# Autodesk Inventor assembly: gearbox_MIR
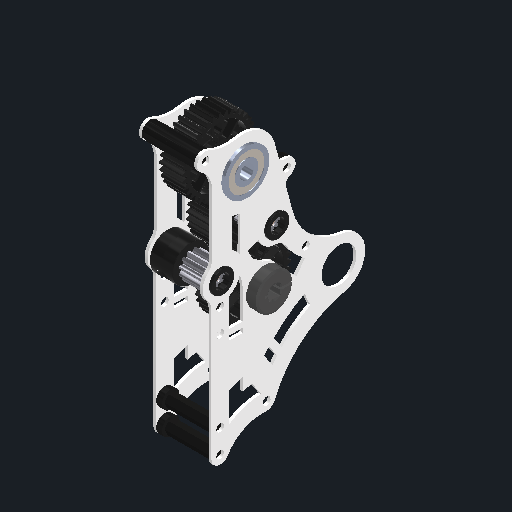
[picture p0: Inventor's stored thumbnail of the model, 512x512]
Saved by Autodesk Inventor 2024 (Build 280153000, 153)
## iProperties
Created: 2023-11-21
Part Number: gearbox_MIR
Document SubType Name: Assembly
Designer: avere
Author: avere
## Documents named in this file (14)
- C:\Users\avere\Documents\rbp_cad\zoomba_v0.1\arm\mirrored_parts\gearbox_MIR.iam
- C:\Users\avere\Documents\rbp_cad\zoomba_v0.1\arm\mirrored_parts\reservoir_mount_MIR.ipt
- C:\Users\avere\Documents\rbp_cad\zoomba_v0.1\arm\mirrored_parts\HS Bushing 0.1250_MIR.ipt
- C:\Users\avere\Documents\rbp_cad\zoomba_v0.1\arm\mirrored_parts\HS 12T Gear, No Insert_MIR.iam
- C:\Users\avere\Documents\rbp_cad\zoomba_v0.1\arm\mirrored_parts\HS 36T Gear, No Insert_MIR.iam
- C:\Users\avere\Documents\rbp_cad\zoomba_v0.1\arm\mirrored_parts\Ball Bearing_MIR.ipt
- C:\Users\avere\Documents\rbp_cad\VEX-CAD-Inventor-1.41\Structure\Standoff\Standoff 1.00.ipt
- C:\Users\avere\Documents\rbp_cad\VEX-CAD-Inventor-1.41\Structure\Standoff.ipt
- C:\Users\avere\Documents\rbp_cad\VEX-CAD-Inventor-1.41\Motion\Spacers\Spacer Nylon .375 OD\NSpacer .375 OD x .125.ipt
- C:\Users\avere\Documents\rbp_cad\VEX-CAD-Inventor-1.41\Motion\Spacers\Spacer Nylon .375 OD.ipt
- C:\Users\avere\Documents\rbp_cad\zoomba_v0.1\arm\mirrored_parts\Low Profile HS Shaft Collar_MIR.ipt
- C:\Users\avere\Documents\rbp_cad\zoomba_v0.1\arm\mirrored_parts\HS Shaft Collar_MIR.ipt
- C:\Users\avere\Documents\rbp_cad\zoomba_v0.1\arm\mirrored_parts\reservoir_mount_inner_MIR.ipt
- C:\Users\avere\Documents\rbp_cad\VEX-CAD-Inventor-1.41\Motion\Spacers\Spacer Nylon .375 OD\NSpacer .375 OD x .500.ipt
## Components (26 placed, 11 different names)
1. reservoir_mount_MIR:1 — Insert:3, Insert:1, Insert:2, Insert:17, Insert:11, Insert:13, Insert:15, Mate:1, Insert:26
2. HS Bushing 0.1250_MIR:1 — Insert:3, Insert:4
3. HS Bushing 0.1250_MIR:2 — Insert:1, Insert:5, Insert:18
4. HS Bushing 0.1250_MIR:3 — Insert:2, Insert:7
5. HS 12T Gear, No Insert_MIR:1 [sub-assembly] — Insert:4
6. HS 12T Gear, No Insert_MIR:2 [sub-assembly] — Insert:6
7. HS 36T Gear, No Insert_MIR:1 [sub-assembly] — Insert:6, Insert:5
8. HS 36T Gear, No Insert_MIR:2 [sub-assembly] — Insert:7, Insert:9
9. HS 12T Gear, No Insert_MIR:3 [sub-assembly] — Insert:9
10. Ball Bearing_MIR:1 — Insert:17
11. Standoff 1.00:1 — Insert:10
12. NSpacer .375 OD x .125:1 — Insert:11, Insert:10
13. NSpacer .375 OD x .125:2 — Insert:13, Insert:21
14. Standoff 1.00:3 — Insert:14
15. NSpacer .375 OD x .125:3 — Insert:14, Insert:15
16. HS 36T Gear, No Insert_MIR:3 [sub-assembly] — Insert:21
17. Low Profile HS Shaft Collar_MIR:1 — Insert:18
18. HS Shaft Collar_MIR:1
19. reservoir_mount_inner_MIR:1 — Mate:1, Insert:20, Insert:24, Insert:25, Insert:26
20. Ball Bearing_MIR:2 — Insert:21, Insert:20
21. NSpacer .375 OD x .500:4
22. NSpacer .375 OD x .500:5 — Insert:21
23. Standoff 1.00:4
24. NSpacer .375 OD x .125:6 — Insert:25
25. Standoff 1.00:5
26. NSpacer .375 OD x .125:7 — Insert:24
## Relationships (25: Insert 24, Mate 1)
- Insert:3: reservoir_mount_MIR:1 ↔ HS Bushing 0.1250_MIR:1
- Insert:1: reservoir_mount_MIR:1 ↔ HS Bushing 0.1250_MIR:2
- Insert:2: reservoir_mount_MIR:1 ↔ HS Bushing 0.1250_MIR:3
- Insert:4 (1.5875 mm): HS Bushing 0.1250_MIR:1 ↔ HS 12T Gear, No Insert_MIR:1
- Insert:6: HS 12T Gear, No Insert_MIR:2 ↔ HS 36T Gear, No Insert_MIR:1
- Insert:5 (1.5875 mm): HS Bushing 0.1250_MIR:2 ↔ HS 36T Gear, No Insert_MIR:1
- Insert:7 (14.2875 mm): HS Bushing 0.1250_MIR:3 ↔ HS 36T Gear, No Insert_MIR:2
- Insert:9: HS 36T Gear, No Insert_MIR:2 ↔ HS 12T Gear, No Insert_MIR:3
- Insert:17: reservoir_mount_MIR:1 ↔ Ball Bearing_MIR:1
- Insert:11: reservoir_mount_MIR:1 ↔ NSpacer .375 OD x .125:1
- Insert:10: Standoff 1.00:1 ↔ NSpacer .375 OD x .125:1
- Insert:13: reservoir_mount_MIR:1 ↔ NSpacer .375 OD x .125:2
- Insert:14: Standoff 1.00:3 ↔ NSpacer .375 OD x .125:3
- Insert:15: reservoir_mount_MIR:1 ↔ NSpacer .375 OD x .125:3
- Insert:18: HS Bushing 0.1250_MIR:2 ↔ Low Profile HS Shaft Collar_MIR:1
- Mate:1: reservoir_mount_MIR:1 ↔ reservoir_mount_inner_MIR:1
- Insert:21: HS 36T Gear, No Insert_MIR:3 ↔ Ball Bearing_MIR:2
- Insert:20: reservoir_mount_inner_MIR:1 ↔ Ball Bearing_MIR:2
- [Insert]: NSpacer .375 OD x .500:4 ↔ NSpacer .375 OD x .500:5
- Insert:21: NSpacer .375 OD x .125:2 ↔ NSpacer .375 OD x .500:5
- [Insert]: Standoff 1.00:4 ↔ NSpacer .375 OD x .125:6
- [Insert]: Standoff 1.00:5 ↔ NSpacer .375 OD x .125:7
- Insert:24: reservoir_mount_inner_MIR:1 ↔ NSpacer .375 OD x .125:7
- Insert:25: reservoir_mount_inner_MIR:1 ↔ NSpacer .375 OD x .125:6
- Insert:26 (28.575 mm): reservoir_mount_MIR:1 ↔ reservoir_mount_inner_MIR:1
## Named parameters: d26_d418_d414 = 0 mm, d23_d26_d418_d414 = 0 mm
